# Autodesk Inventor assembly: tower 3_1
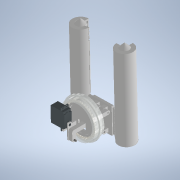
[picture p0: Inventor's stored thumbnail of the model, 180x180]
Saved by Autodesk Inventor 2020.1 (Build 241239000, 239)
## iProperties
Created: 2022-04-03
Part Number: tower 3_1
Document SubType Name: Assembly
Designer: User
Author: User
## Documents named in this file (7)
- D:\GitHub\TANK\3D-turret\tower 3_1.iam
- D:\GitHub\TANK\3D-turret\tower 3.iam
- D:\GitHub\TANK\3D-turret\колено для сервы.ipt
- D:\GitHub\TANK\3D-turret\подшипник.iam
- D:\GitHub\TANK\3D-turret\MG996R.ipt
- D:\GitHub\TANK\3D-turret\лапка сервы.ipt
- D:\GitHub\TANK\3D-turret\болт м4 20мм.ipt
## Components (6 placed, 6 different names)
1. tower 3:1 [sub-assembly] — Вставка:3, Вставка:5
2. подшипник:1 [sub-assembly] — Вставка:3, Угол:3, Жесткий:1
3. MG996R:1 — Угол:3, Жесткий:1, Вставка:4
4. лапка сервы:1 — Вставка:4, Вставка:6
5. колено для сервы:1 — Вставка:5, Совмещение:1
6. BS 4183 Винты и гайки крепежные мелкие. Метрическая серия - метрическая M4 x 20:1 — Вставка:6, Совмещение:1
## Relationships (7: Insert 4, Angle 1, WeldJoint 1, Mate 1)
- Вставка:3 [Insert]: tower 3:1 ↔ подшипник:1
- Угол:3 [Angle] (0 deg): подшипник:1 ↔ MG996R:1
- Жесткий:1 [WeldJoint]: подшипник:1 ↔ MG996R:1
- Вставка:4 [Insert]: MG996R:1 ↔ лапка сервы:1
- Вставка:5 [Insert]: tower 3:1 ↔ колено для сервы:1
- Вставка:6 [Insert]: лапка сервы:1 ↔ BS 4183 Винты и гайки крепежные мелкие. Метрическая серия - метрическая M4 x 20:1
- Совмещение:1 [Mate]: колено для сервы:1 ↔ BS 4183 Винты и гайки крепежные мелкие. Метрическая серия - метрическая M4 x 20:1
